# Autodesk Inventor assembly: DelrinWheel_MIR
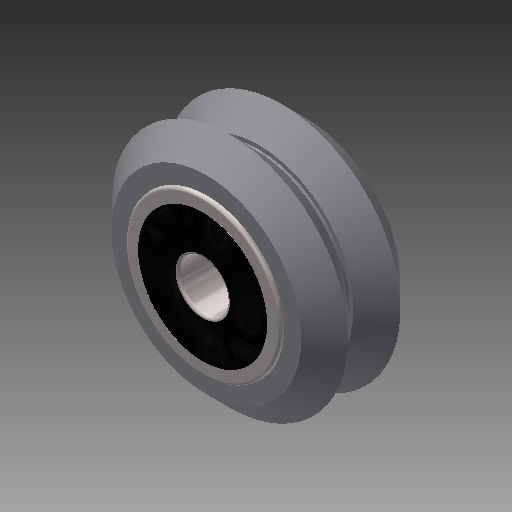
[picture p0: Inventor's stored thumbnail of the model, 512x512]
Saved by Autodesk Inventor 2018 (Build 220112000, 112)
## iProperties
Created: 2016-07-20
Part Number: DelrinWheel_MIR
Document SubType Name: Assembly
Designer: User
Author: User
## Documents named in this file (4)
- C:\Users\Dan\OneDrive\SL-Inventor\The Beast v1.2 PackandGo\Workspaces\Workspace\DelrinWheel_MIR.iam
- C:\Users\Dan\OneDrive\SL-Inventor\The Beast v1.2 PackandGo\Workspaces\Workspace\dELRIN_MIR1.ipt
- C:\Users\Dan\OneDrive\SL-Inventor\The Beast v1.2 PackandGo\Workspaces\Workspace\SKF 625_MIR1.ipt
- C:\Users\Dan\OneDrive\SL-Inventor\The Beast v1.2 PackandGo\Workspaces\Workspace\SKF 625_CPY_MIR1.ipt
## Components (3 placed, 3 different names)
1. dELRIN_MIR1:1 — Mate:2, Mate:1, Mate:4, Mate:3
2. SKF 625_MIR1:1 — Mate:2, Mate:1
3. SKF 625_CPY_MIR1:1 — Mate:4, Mate:3
## Relationships (4: Mate 4)
- Mate:2: dELRIN_MIR1:1 ↔ SKF 625_MIR1:1
- Mate:1: dELRIN_MIR1:1 ↔ SKF 625_MIR1:1
- Mate:4: dELRIN_MIR1:1 ↔ SKF 625_CPY_MIR1:1
- Mate:3: dELRIN_MIR1:1 ↔ SKF 625_CPY_MIR1:1
